# Autodesk Inventor assembly: Assembly1
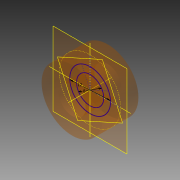
[picture p0: Inventor's stored thumbnail of the model, 180x180]
Saved by Autodesk Inventor 2018.2 (Build 222227000, 227)
## iProperties
Created: 2018-02-28
Part Number: Assembly1
Document SubType Name: Assembly
Designer: Rus
Author: Rus
## Documents named in this file (4)
- E:\Libraries\3D Objects\Longboard\Spacer and Rings\Assembly1.iam
- E:\Libraries\3D Objects\Longboard\Spacer and Rings\Spacer.ipt
- E:\Libraries\3D Objects\Longboard\Spacer and Rings\Washer.ipt
- E:\Libraries\3D Objects\Longboard\Inside Wheels Limits\V0\Inside Wheel Limits.ipt
## Components (3 placed, 3 different names)
1. Spacer:1 — Angle:1, Tangent:1, Flush:1
2. Washer:1
3. Inside Wheel Limits:1 — Angle:1, Tangent:1, Flush:1
## Relationships (3: Angle 1, Tangent 1, Flush 1)
- Angle:1 (0 deg): Spacer:1 ↔ Inside Wheel Limits:1
- Tangent:1: Spacer:1 ↔ Inside Wheel Limits:1
- Flush:1: Spacer:1 ↔ Inside Wheel Limits:1
